# Autodesk Inventor assembly: EPS
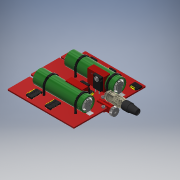
[picture p0: Inventor's stored thumbnail of the model, 180x180]
Saved by Autodesk Inventor 2018 (Build 220112000, 112)
## iProperties
Created: 2018-05-29
Part Number: EPS
Document SubType Name: Assembly
Designer: Bradley
Mass: 141.712 g
Surface Area: 416.928 cm^2
Volume: 50.0199 cm^3
Density: 2.83312 g/cm^3
Author: Bradley
## Documents named in this file (20)
- C:\Users\Bradley\Documents\GitHub\CougSat1-Hardware\CougSat1-PowerBoard\CADModel\Native\EPS.iam
- C:\Users\Bradley\Documents\GitHub\CougSat1-Hardware\CougSat1-PowerBoard\CADModel\Native\EPS_PCB.ipt
- C:\Users\Bradley\Documents\GitHub\Resources\ComponentModels\Electronics\Battery_18650.ipt
- C:\Users\Bradley\Documents\GitHub\Resources\ComponentModels\Connectors\PicoLock-J-7.ipt
- C:\Users\Bradley\Documents\GitHub\Resources\ComponentModels\Connectors\PicoLock-J-4.ipt
- C:\Users\Bradley\Documents\GitHub\Resources\ComponentModels\Connectors\PicoLock-P-4.ipt
- C:\Users\Bradley\Documents\GitHub\Resources\ComponentModels\Connectors\PicoLock-P-7.ipt
- C:\Users\Bradley\Documents\GitHub\CougSat1-Hardware\CougSat1-PowerBoard\CADModel\Native\EPS_RBFPinHolder.ipt
- C:\Users\Bradley\Documents\GitHub\Resources\ComponentModels\Electronics\Resistor_TH-TO220.ipt
- C:\Users\Bradley\Documents\GitHub\CougSat1-Hardware\CougSat1-PowerBoard\CADModel\Native\EPS_BatteryTab.ipt
- C:\Users\Bradley\Documents\GitHub\CougSat1-Hardware\CougSat1-PowerBoard\CADModel\Native\EPS_BatteyTie.ipt
- C:\Users\Bradley\Documents\GitHub\Resources\ComponentModels\Connectors\HR10A-7R-4P.ipt
- C:\Users\Bradley\Documents\GitHub\Resources\ComponentModels\Connectors\HR10A-7P-4S.ipt
- C:\Users\Bradley\Documents\GitHub\Resources\ComponentModels\Fasteners\Nut_M8x0.5_2mm.ipt
- C:\Users\Bradley\Documents\GitHub\Resources\ComponentModels\Connectors\SMD2.54-1x06-R.ipt
- C:\Users\Bradley\Documents\GitHub\CougSat1-Hardware\CougSat1-PowerBoard\CADModel\Native\EPS_BatteryHeatsink.ipt
- C:\Users\Bradley\Documents\GitHub\Resources\ComponentModels\Fasteners\Bolt_M3x0.35_6mm_BH.ipt
- C:\Users\Bradley\Documents\GitHub\Resources\ComponentModels\Fasteners\BoltThumb_M4x0.7_19mm-SHD_5mm.ipt
- C:\Users\Bradley\Documents\GitHub\Resources\ComponentModels\Fasteners\Bolt_M2x0.4_4mm_SH.ipt
- C:\Users\Bradley\Documents\GitHub\Resources\ComponentModels\Electronics\Switch_Micro-SMT.ipt
## Components (38 placed, 19 different names)
1. EPS_BatteryHeatsink:1 — Insert:15, Mate:545
2. EPS_BatteryHeatsink:2 — Mate:544, Insert:19
3. EPS_PCB:1 — Flush:1, Flush:2, Mate:14, Mate:15, Mate:16, Mate:17, Mate:18, Insert:4, Insert:9, Mate:22, Mate:23, Mate:24, Mate:25, Mate:26, Mate:35, Mate:36, Mate:37, Mate:38, Mate:45, Mate:46, Mate:47, Mate:48, Mate:49, Mate:50, Mate:51, Mate:52, Flush:23, Mate:55, Mate:56, Mate:57, Flush:28, Mate:62, Insert:21, Insert:22, Mate:546, Flush:31
4. EPS_RBFPinHolder:1 — Insert:4, Insert:9, Insert:20
5. HR10A-7R-4P:1 — Insert:14, Flush:20, Mate:53, Flush:22, Mate:54, Mate:55
6. HR10A-7P-4S:1 — Insert:14, Flush:20
7. PicoLock-J-4:1 — Flush:5, Mate:4, Mate:5, Mate:18, Mate:20, Mate:56
8. PicoLock-J-4:2 — Mate:62, Mate:63, Mate:64
9. PicoLock-J-7:1 — Flush:6, Mate:6, Mate:7, Mate:14, Flush:14, Flush:24
10. PicoLock-J-7:2 — Mate:15, Flush:15, Flush:25
11. PicoLock-J-7:3 — Mate:16, Flush:14, Mate:23, Flush:26
12. PicoLock-J-7:4 — Mate:17, Flush:15, Mate:24, Flush:27
13. PicoLock-P-4:1 — Flush:5, Mate:4, Mate:5
14. PicoLock-P-4:2
15. PicoLock-P-7:1 — Flush:6, Mate:6, Mate:7
16. PicoLock-P-7:2
17. PicoLock-P-7:3
18. PicoLock-P-7:4
19. SMD2.54-1x06-R:1 — Mate:57, Mate:58, Flush:28
20. Battery_18650:1 — Flush:1, Flush:4, Mate:30, Mate:32, Mate:33, Mate:39, Flush:18, Mate:41, Mate:42, Mate:544
21. Battery_18650:2 — Flush:2, Flush:3, Mate:29, Mate:31, Mate:34, Mate:40, Flush:19, Mate:43, Mate:44, Mate:545
22. EPS_BatteryTab:1 — Mate:32, Mate:38, Mate:39
23. EPS_BatteryTab:2 — Mate:33, Mate:36, Flush:18
24. EPS_BatteryTab:3 — Mate:31, Mate:37, Mate:40
25. EPS_BatteryTab:4 — Mate:34, Mate:35, Flush:19
26. Resistor_TH-TO220:1 — Mate:22, Mate:25, Mate:28, Flush:29, Insert:18, Insert:19
27. Resistor_TH-TO220:2 — Mate:26, Mate:28, Mate:59, Insert:15, Insert:17
28. Switch_Micro-SMT:1 — Mate:546, Flush:31, Mate:547
29. Bolt_M2x0.4_4mm_SH:1 — Insert:21
30. Bolt_M2x0.4_4mm_SH:2 — Insert:22
31. Bolt_M3x0.35_6mm_BH:1 — Insert:17
32. Bolt_M3x0.35_6mm_BH:2 — Insert:18
33. EPS_BatteyTie:1 — Mate:41, Mate:47, Mate:49
34. EPS_BatteyTie:2 — Mate:42, Mate:48, Mate:50
35. EPS_BatteyTie:3 — Mate:43, Mate:45, Mate:51
36. EPS_BatteyTie:4 — Mate:44, Mate:46, Mate:52
37. Nut_M8x0.5_2mm:1 — Mate:54, Flush:23
38. BoltThumb_M4x0.7_19mm-SHD_5mm:1 — Insert:20
## Relationships (96: Mate 62, Flush 24, Insert 10)
- Flush:1 (-9.15 mm): EPS_PCB:1 ↔ Battery_18650:1
- Flush:2 (-9.15 mm): EPS_PCB:1 ↔ Battery_18650:2
- Flush:3 (-50 mm): Battery_18650:2
- Flush:4 (-50 mm): Battery_18650:1
- Flush:5: PicoLock-J-4:1 ↔ PicoLock-P-4:1
- Mate:4: PicoLock-J-4:1 ↔ PicoLock-P-4:1
- Mate:5 (0.025 mm): PicoLock-J-4:1 ↔ PicoLock-P-4:1
- Flush:6: PicoLock-J-7:1 ↔ PicoLock-P-7:1
- Mate:6: PicoLock-J-7:1 ↔ PicoLock-P-7:1
- Mate:7 (0.025 mm): PicoLock-J-7:1 ↔ PicoLock-P-7:1
- [Flush]: PicoLock-J-7:2 ↔ PicoLock-P-7:2
- [Mate]: PicoLock-J-7:2 ↔ PicoLock-P-7:2
- [Mate] (0.025 mm): PicoLock-J-7:2 ↔ PicoLock-P-7:2
- [Flush]: PicoLock-J-7:3 ↔ PicoLock-P-7:3
- [Mate]: PicoLock-J-7:3 ↔ PicoLock-P-7:3
- [Mate] (0.025 mm): PicoLock-J-7:3 ↔ PicoLock-P-7:3
- [Flush]: PicoLock-J-7:4 ↔ PicoLock-P-7:4
- [Mate]: PicoLock-J-7:4 ↔ PicoLock-P-7:4
- [Mate] (0.025 mm): PicoLock-J-7:4 ↔ PicoLock-P-7:4
- Mate:14: EPS_PCB:1 ↔ PicoLock-J-7:1
- Mate:15: EPS_PCB:1 ↔ PicoLock-J-7:2
- Mate:16: EPS_PCB:1 ↔ PicoLock-J-7:3
- Mate:17: EPS_PCB:1 ↔ PicoLock-J-7:4
- Mate:18: EPS_PCB:1 ↔ PicoLock-J-4:1
- Flush:14: PicoLock-J-7:1 ↔ PicoLock-J-7:3
- Flush:15: PicoLock-J-7:2 ↔ PicoLock-J-7:4
- Insert:4: EPS_PCB:1 ↔ EPS_RBFPinHolder:1
- Insert:9: EPS_PCB:1 ↔ EPS_RBFPinHolder:1
- Mate:20: PicoLock-J-4:1
- Mate:22: EPS_PCB:1 ↔ Resistor_TH-TO220:1
- Mate:23 (-30 mm): EPS_PCB:1 ↔ PicoLock-J-7:3
- Mate:24 (-55 mm): EPS_PCB:1 ↔ PicoLock-J-7:4
- Mate:25 (-66 mm): EPS_PCB:1 ↔ Resistor_TH-TO220:1
- Mate:26: EPS_PCB:1 ↔ Resistor_TH-TO220:2
- Mate:28: Resistor_TH-TO220:1 ↔ Resistor_TH-TO220:2
- Mate:29 (-21 mm): Battery_18650:2
- Mate:30 (21 mm): Battery_18650:1
- Mate:31: Battery_18650:2 ↔ EPS_BatteryTab:3
- Mate:32: Battery_18650:1 ↔ EPS_BatteryTab:1
- Mate:33: Battery_18650:1 ↔ EPS_BatteryTab:2
- Mate:34: Battery_18650:2 ↔ EPS_BatteryTab:4
- Mate:35: EPS_PCB:1 ↔ EPS_BatteryTab:4
- Mate:36: EPS_PCB:1 ↔ EPS_BatteryTab:2
- Mate:37: EPS_PCB:1 ↔ EPS_BatteryTab:3
- Mate:38: EPS_PCB:1 ↔ EPS_BatteryTab:1
- Mate:39: Battery_18650:1 ↔ EPS_BatteryTab:1
- Flush:18: Battery_18650:1 ↔ EPS_BatteryTab:2
- Mate:40: Battery_18650:2 ↔ EPS_BatteryTab:3
- Flush:19: Battery_18650:2 ↔ EPS_BatteryTab:4
- Mate:41: Battery_18650:1 ↔ EPS_BatteyTie:1
- Mate:42: Battery_18650:1 ↔ EPS_BatteyTie:2
- Mate:43: Battery_18650:2 ↔ EPS_BatteyTie:3
- Mate:44: Battery_18650:2 ↔ EPS_BatteyTie:4
- Mate:45: EPS_PCB:1 ↔ EPS_BatteyTie:3
- Mate:46: EPS_PCB:1 ↔ EPS_BatteyTie:4
- Mate:47: EPS_PCB:1 ↔ EPS_BatteyTie:1
- Mate:48: EPS_PCB:1 ↔ EPS_BatteyTie:2
- Mate:49: EPS_PCB:1 ↔ EPS_BatteyTie:1
- Mate:50: EPS_PCB:1 ↔ EPS_BatteyTie:2
- Mate:51: EPS_PCB:1 ↔ EPS_BatteyTie:3
- Mate:52: EPS_PCB:1 ↔ EPS_BatteyTie:4
- Insert:14: HR10A-7R-4P:1 ↔ HR10A-7P-4S:1
- Flush:20: HR10A-7R-4P:1 ↔ HR10A-7P-4S:1
- Mate:53 (13 mm): HR10A-7R-4P:1
- Flush:22: HR10A-7R-4P:1
- Mate:54: HR10A-7R-4P:1 ↔ Nut_M8x0.5_2mm:1
- Flush:23: EPS_PCB:1 ↔ Nut_M8x0.5_2mm:1
- Mate:55 (1.7 mm): EPS_PCB:1 ↔ HR10A-7R-4P:1
- Mate:56 (-33 mm): EPS_PCB:1 ↔ PicoLock-J-4:1
- Flush:24 (-36.75 mm): PicoLock-J-7:1
- Flush:25 (-36.75 mm): PicoLock-J-7:2
- Flush:26 (36.75 mm): PicoLock-J-7:3
- Flush:27 (36.75 mm): PicoLock-J-7:4
- Mate:57: EPS_PCB:1 ↔ SMD2.54-1x06-R:1
- Mate:58 (6.35 mm): SMD2.54-1x06-R:1
- Flush:28 (50 mm): EPS_PCB:1 ↔ SMD2.54-1x06-R:1
- Mate:59 (-9.8 mm): Resistor_TH-TO220:2
- Flush:29 (-9.8 mm): Resistor_TH-TO220:1
- [Flush]: PicoLock-J-4:2 ↔ PicoLock-P-4:2
- [Mate]: PicoLock-J-4:2 ↔ PicoLock-P-4:2
- [Mate] (0.025 mm): PicoLock-J-4:2 ↔ PicoLock-P-4:2
- Mate:62: EPS_PCB:1 ↔ PicoLock-J-4:2
- Mate:63 (85.3 mm): PicoLock-J-4:2
- Mate:64 (43.5 mm): PicoLock-J-4:2
- Insert:15: EPS_BatteryHeatsink:1 ↔ Resistor_TH-TO220:2
- Mate:544: EPS_BatteryHeatsink:2 ↔ Battery_18650:1
- Mate:545: EPS_BatteryHeatsink:1 ↔ Battery_18650:2
- Insert:17: Resistor_TH-TO220:2 ↔ Bolt_M3x0.35_6mm_BH:1
- Insert:18: Resistor_TH-TO220:1 ↔ Bolt_M3x0.35_6mm_BH:2
- Insert:19: EPS_BatteryHeatsink:2 ↔ Resistor_TH-TO220:1
- Insert:20: EPS_RBFPinHolder:1 ↔ BoltThumb_M4x0.7_19mm-SHD_5mm:1
- Insert:21: EPS_PCB:1 ↔ Bolt_M2x0.4_4mm_SH:1
- Insert:22: EPS_PCB:1 ↔ Bolt_M2x0.4_4mm_SH:2
- Mate:546: EPS_PCB:1 ↔ Switch_Micro-SMT:1
- Flush:31 (-6.05 mm): EPS_PCB:1 ↔ Switch_Micro-SMT:1
- Mate:547 (8.9 mm): Switch_Micro-SMT:1
## Named parameters: d15_d12 = 0 mm, d16_d13 = 0 mm, d17_d14 = 0.025 mm, d18_d12 = 0 mm, d19_d13 = 0 mm, d20_d14 = 0.025 mm, d21_d12 = 0 mm, d22_d13 = 0 mm, d23_d14 = 0.025 mm, d105_d9 = 0 mm, d106_d10 = 0 mm, d107_d11 = 0.025 mm
